# Autodesk Inventor assembly: NEMA17_GT2B5W10
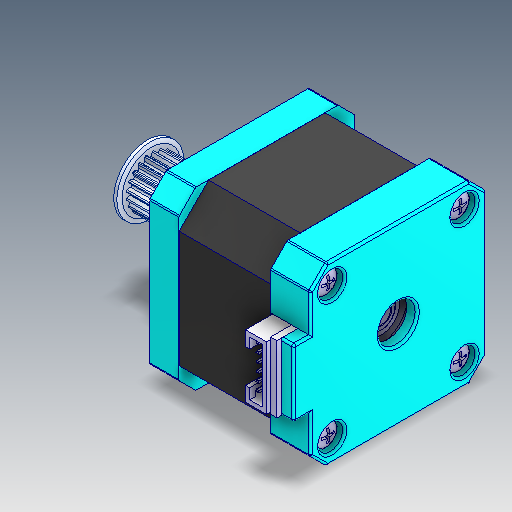
[picture p0: Inventor's stored thumbnail of the model, 512x512]
Saved by Autodesk Inventor 2020 (Build 240168000, 168)
## iProperties
Created: 2020-03-26
Part Number: NEMA17_GT2B5W10
Document SubType Name: Assembly
Designer: chitl
Author: chitl
## Documents named in this file (3)
- C:\Users\chitl\Desktop\CNC-Drawing-Robot\Inventor Files\NEMA Motor\NEMA17_GT2B5W10.iam
- C:\Users\chitl\Desktop\CNC-Drawing-Robot\Inventor Files\NEMA Motor\NEMA17.ipt
- C:\Users\chitl\Desktop\CNC-Drawing-Robot\Inventor Files\Timing Pulley\gt2-timing-belt-pulley-1.snapshot.2\GT2\GT2.ipt
## Components (2 placed, 2 different names)
1. NEMA17:1 — Mate:1
2. GT2:1 — Mate:1
## Relationships (1: Mate 1)
- Mate:1: NEMA17:1 ↔ GT2:1
